# Autodesk Inventor assembly: dribler_v2
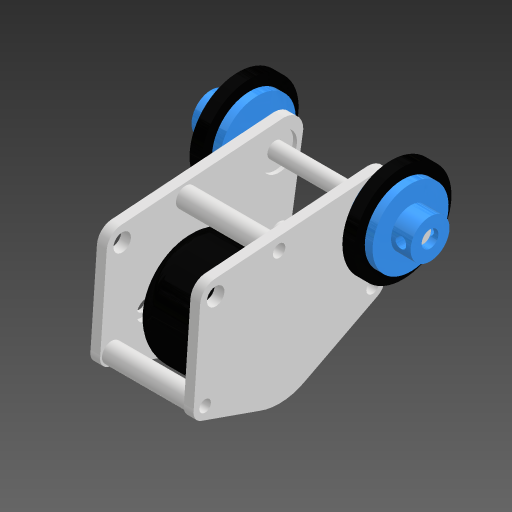
[picture p0: Inventor's stored thumbnail of the model, 512x512]
Saved by Autodesk Inventor 2023 (Build 270158000, 158)
## iProperties
Created: 2025-09-24
Part Number: dribler_v2
Document SubType Name: Assembly
Designer: daa
Author: daa
## Documents named in this file (9)
- C:\Users\daa\Documents\DASH_V2\Dribler_v2\dribler_v2.iam
- C:\Users\daa\Documents\DASH_V2\Dribler_v2\drib_lef.ipt
- C:\Users\daa\Documents\DASH_V2\Dribler_v2\drib_rig.ipt
- C:\Users\daa\Documents\DASH_V2\Dribler_v2\motor_c2822.ipt
- C:\Users\daa\Documents\DASH_V2\Dribler_v2\rack.ipt
- C:\Users\daa\Documents\DASH_V2\Dribler_v2\bearing.ipt
- C:\Users\daa\Documents\DASH_V2\Dribler_v2\axis.ipt
- C:\Users\daa\Documents\DASH_V2\Dribler_v2\koleso_left.ipt
- C:\Users\daa\Documents\DASH_V2\Dribler_v2\Деталь1222.ipt
## Components (13 placed, 8 different names)
1. drib_lef:1 — Совмещение:1, С поворотом:5
2. drib_rig:1 — С поворотом:1, С поворотом:2, С поворотом:3, С поворотом:4, С поворотом:6
3. rack:1 — С поворотом:3
4. rack:2 — С поворотом:2
5. rack:3 — С поворотом:1, Совмещение:1
6. bearing:1 — С поворотом:4
7. bearing:2 — С поворотом:5, Жесткий:2
8. axis:1 — Жесткий:2, Жесткий:3, Жесткий:4
9. koleso_left:1 — Жесткий:3, С поворотом:8
10. koleso_left:2 — Жесткий:4, С поворотом:7
11. motor_c2822:1 — С поворотом:6
12. Деталь1222:1 — С поворотом:7
13. Деталь1222:2 — С поворотом:8
## Relationships (12: RevoluteJoint 8, WeldJoint 3, Mate 1)
- С поворотом:1 [RevoluteJoint]: drib_rig:1 ↔ rack:3
- С поворотом:2 [RevoluteJoint]: drib_rig:1 ↔ rack:2
- С поворотом:3 [RevoluteJoint]: drib_rig:1 ↔ rack:1
- Совмещение:1 [Mate]: drib_lef:1 ↔ rack:3
- С поворотом:4 [RevoluteJoint] (-1.5 mm): drib_rig:1 ↔ bearing:1
- С поворотом:5 [RevoluteJoint] (1.5 mm): drib_lef:1 ↔ bearing:2
- Жесткий:2 [WeldJoint] (-14.5 mm): bearing:2 ↔ axis:1
- С поворотом:6 [RevoluteJoint] (6 mm): drib_rig:1 ↔ motor_c2822:1
- Жесткий:3 [WeldJoint] (-14 mm): axis:1 ↔ koleso_left:1
- Жесткий:4 [WeldJoint] (-11.75 mm): axis:1 ↔ koleso_left:2
- С поворотом:7 [RevoluteJoint]: koleso_left:2 ↔ Деталь1222:1
- С поворотом:8 [RevoluteJoint]: koleso_left:1 ↔ Деталь1222:2
